# Autodesk Inventor assembly: Rod Holder D
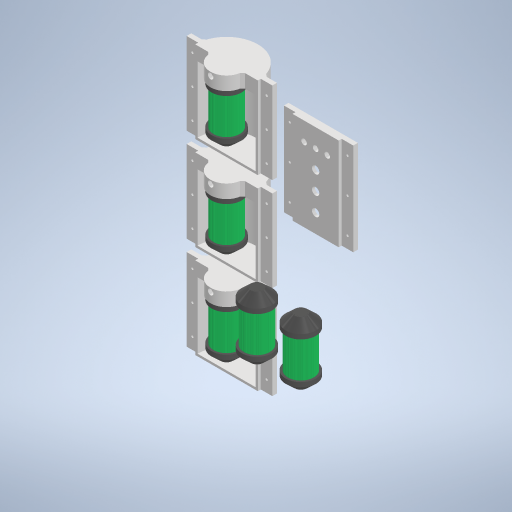
[picture p0: Inventor's stored thumbnail of the model, 512x512]
Saved by Autodesk Inventor 2024 (Build 280153020, 153B)
## iProperties
Created: 2023-08-02
Part Number: Rod Holder D
Document SubType Name: Assembly
Designer: torban
Author: torban
## Documents named in this file (4)
- D:\GIT\CIRC-2023-Night-Task-HW-SW\CAD\Reactor Control Panel\Rod Holder D.iam
- D:\GIT\CIRC-2023-Night-Task-HW-SW\CAD\Reactor\Reactor\Full.iam
- D:\GIT\CIRC-2023-Night-Task-HW-SW\CAD\Reactor Control Panel\Faceplate.ipt
- D:\GIT\CIRC-2023-Night-Task-HW-SW\CAD\Reactor Module\Reactor Module\Reactor Rod Holder Positions.iam
## Components (5 placed, 3 different names)
1. Full:1 [sub-assembly] — Mate:1, Flush:2, Flush:3, Mate:4
2. Full:2 [sub-assembly] — Mate:2, Flush:1, Flush:4, Flush:5, Flush:6
3. Full:3 [sub-assembly] — Mate:1, Mate:2, Flush:1, Flush:2, Flush:3, Flush:4, Mate:3
4. Faceplate:1 — Flush:5, Mate:3, Flush:6
5. Reactor Rod Holder Positions:1 [sub-assembly] — Mate:4
## Relationships (10: Flush 6, Mate 4)
- Mate:1 (25 mm): Full:1 ↔ Full:3
- Mate:2 (25 mm): Full:2 ↔ Full:3
- Flush:1: Full:2 ↔ Full:3
- Flush:2: Full:1 ↔ Full:3
- Flush:3: Full:1 ↔ Full:3
- Flush:4: Full:2 ↔ Full:3
- Flush:5: Full:2 ↔ Faceplate:1
- Mate:3 (25 mm): Full:3 ↔ Faceplate:1
- Flush:6: Full:2 ↔ Faceplate:1
- Mate:4: Full:1 ↔ Reactor Rod Holder Positions:1
